# Autodesk Inventor assembly: Сборка штурвал
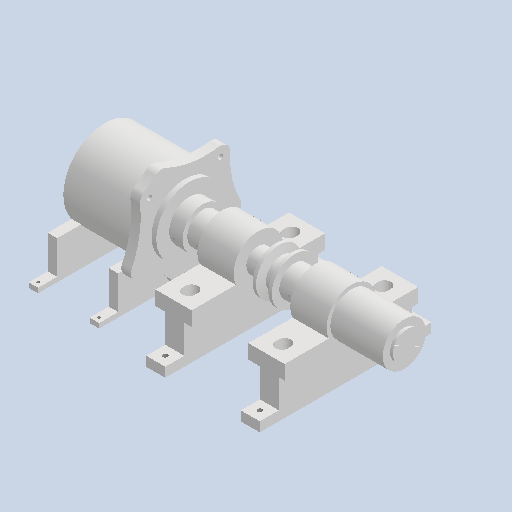
[picture p0: Inventor's stored thumbnail of the model, 512x512]
Saved by Autodesk Inventor 2023 (Build 270158000, 158)
## iProperties
Created: 2022-05-01
Part Number: Сборка штурвал
Document SubType Name: Assembly
Designer: User
Author: User
## Documents named in this file (11)
- D:\Стойка\VR-simulator-3D-models\Механизм\Сборка механизма штурвала.iam
- D:\Стойка\VR-simulator-3D-models\Архив\Маховик.ipt
- D:\Стойка\VR-simulator-3D-models\Механизм\Вал.ipt
- D:\Стойка\VR-simulator-3D-models\Механизм\Стена 16 мм отверстие.ipt
- D:\Стойка\VR-simulator-3D-models\Механизм\Подшипник с лапками.ipt
- D:\Стойка\VR-simulator-3D-models\Механизм\Подставка подшипника.ipt
- D:\Стойка\VR-simulator-3D-models\Механизм\Шкив малый.ipt
- D:\Стойка\VR-simulator-3D-models\Механизм\Болт маховика.ipt
- D:\Стойка\VR-simulator-3D-models\Механизм\Двигатель.ipt
- D:\Стойка\VR-simulator-3D-models\Механизм\Муфта штурвал, двигатель.ipt
- D:\Стойка\VR-simulator-3D-models\Механизм\Мотор стенка.ipt
## Components (14 placed, 10 different names)
1. Стена 16 мм отверстие:1 — Заподлицо:1
2. Стена 16 мм отверстие:2 — Заподлицо:1
3. Подшипник с лапками:1 — Цилиндрический:22, Заподлицо:6, Совмещение:88
4. Подшипник с лапками:2 — Цилиндрический:22, Совмещение:21, Заподлицо:3, Совмещение:75, Совмещение:89
5. Вал:1 — Совмещение:21, Совмещение:59, Совмещение:72, Совмещение:73, Совмещение:76, Совмещение:90
6. Маховик:1 — Совмещение:89, Совмещение:90, Совмещение:91, Совмещение:92
7. Подставка подшипника:1 — Заподлицо:6
8. Подставка подшипника:2 — Заподлицо:3, Совмещение:75
9. Шкив малый:1 — Совмещение:59, Совмещение:76
10. Болт маховика:1 — Совмещение:91, Совмещение:92
11. Двигатель:1 — Совмещение:70, Совмещение:71, Совмещение:73, Совмещение:78, Совмещение:79, Совмещение:82, Совмещение:83, Заподлицо:11
12. Муфта штурвал, двигатель:1 — Совмещение:70, Совмещение:71, Совмещение:72, Совмещение:88
13. Мотор стенка:1 — Совмещение:79, Совмещение:82, Совмещение:83
14. Мотор стенка:2 — Совмещение:78, Заподлицо:11
## Relationships (22: Mate 17, Flush 4, CylindricalJoint 1)
- Заподлицо:1 [Flush]: Стена 16 мм отверстие:1 ↔ Стена 16 мм отверстие:2
- Цилиндрический:22 [CylindricalJoint]: Подшипник с лапками:1 ↔ Подшипник с лапками:2
- Совмещение:21 [Mate]: Подшипник с лапками:2 ↔ Вал:1
- Заподлицо:3 [Flush]: Подшипник с лапками:2 ↔ Подставка подшипника:2
- Заподлицо:6 [Flush]: Подшипник с лапками:1 ↔ Подставка подшипника:1
- Совмещение:59 [Mate]: Вал:1 ↔ Шкив малый:1
- Совмещение:70 [Mate]: Двигатель:1 ↔ Муфта штурвал, двигатель:1
- Совмещение:71 [Mate]: Двигатель:1 ↔ Муфта штурвал, двигатель:1
- Совмещение:72 [Mate]: Вал:1 ↔ Муфта штурвал, двигатель:1
- Совмещение:73 [Mate]: Вал:1 ↔ Двигатель:1
- Совмещение:75 [Mate]: Подшипник с лапками:2 ↔ Подставка подшипника:2
- Совмещение:76 [Mate]: Вал:1 ↔ Шкив малый:1
- Совмещение:78 [Mate]: Двигатель:1 ↔ Мотор стенка:2
- Совмещение:79 [Mate]: Двигатель:1 ↔ Мотор стенка:1
- Совмещение:82 [Mate]: Двигатель:1 ↔ Мотор стенка:1
- Совмещение:83 [Mate]: Двигатель:1 ↔ Мотор стенка:1
- Заподлицо:11 [Flush]: Двигатель:1 ↔ Мотор стенка:2
- Совмещение:88 [Mate]: Подшипник с лапками:1 ↔ Муфта штурвал, двигатель:1
- Совмещение:89 [Mate]: Подшипник с лапками:2 ↔ Маховик:1
- Совмещение:90 [Mate]: Вал:1 ↔ Маховик:1
- Совмещение:91 [Mate]: Маховик:1 ↔ Болт маховика:1
- Совмещение:92 [Mate]: Маховик:1 ↔ Болт маховика:1
